# Autodesk Inventor assembly: Grundstück
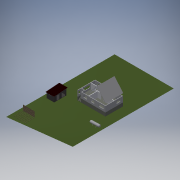
[picture p0: Inventor's stored thumbnail of the model, 180x180]
Saved by Autodesk Inventor 2017 (Build 210142000, 142)
## iProperties
Created: 2017-05-10
Part Number: Grundstück
Document SubType Name: Assembly
Designer: Fake
Author: Fake
## Documents named in this file (6)
- C:\Users\Fake\Documents\Inventor\Oli_Grundstück\Grundstück.iam
- C:\Users\Fake\Documents\Inventor\Oli_Grundstück\Grundstück.ipt
- C:\Users\Fake\Documents\Inventor\Oli_Grundstück\Schuppen.iam
- C:\Users\Fake\Documents\Inventor\Oli_Grundstück\Haus.iam
- C:\Users\Fake\Documents\Inventor\Oli_Grundstück\Gascontainer.ipt
- C:\Users\Fake\Documents\Inventor\Oli_Grundstück\Blockhaus.iam
## Components (5 placed, 5 different names)
1. Grundstück:1 — Passend:1, Passend:2, Passend:3, Passend:4, Passend:5
2. Gascontainer:1 — Passend:3
3. Blockhaus:1 [sub-assembly] — Passend:4
4. Schuppen:1 [sub-assembly] — Passend:1
5. Haus:1 [sub-assembly] — Passend:2, Passend:5
## Relationships (5: Mate 5)
- Passend:1 [Mate]: Grundstück:1 ↔ Schuppen:1
- Passend:2 [Mate]: Grundstück:1 ↔ Haus:1
- Passend:3 [Mate]: Grundstück:1 ↔ Gascontainer:1
- Passend:4 [Mate]: Grundstück:1 ↔ Blockhaus:1
- Passend:5 [Mate] (4000 mm): Grundstück:1 ↔ Haus:1
